# Autodesk Inventor assembly: Lid Connected To Body
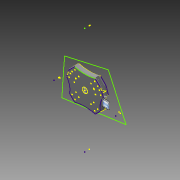
[picture p0: Inventor's stored thumbnail of the model, 180x180]
Saved by Autodesk Inventor 2014 (Build 180170000, 170)
## iProperties
Created: 2014-03-02
Part Number: Lid Connected To Body
Document SubType Name: Assembly
Designer: Isaac
Author: Isaac
## Documents named in this file (3)
- C:\Everything Quadcopter\Quadcopter Design\MakerBot Upload Files\Lid Connected To Body.iam
- C:\Everything Quadcopter\Quadcopter Design\Refined DeadCat X Body (V2).ipt
- C:\Everything Quadcopter\Quadcopter Design\MakerBot Upload Files\Main Body Lid.ipt
## Components (2 placed, 2 different names)
1. Refined DeadCat X Body (V2):1 — Rigid:1
2. Main Body Lid:1 — Rigid:1
## Relationships (1: WeldJoint 1)
- Rigid:1 [WeldJoint]: Refined DeadCat X Body (V2):1 ↔ Main Body Lid:1
